# Autodesk Inventor assembly: aftServoSectionAssembly0
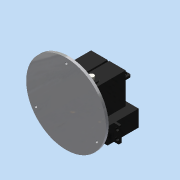
[picture p0: Inventor's stored thumbnail of the model, 180x180]
Saved by Autodesk Inventor 2017 (Build 210142000, 142)
## iProperties
Created: 2016-10-29
Part Number: aftServoSectionAssembly0
Document SubType Name: Assembly
Designer: techn
Author: techn
## Documents named in this file (4)
- D:\OneDrive\Documents\Other Projects\Submarine\CAD\midships\AftServoSection\aftServoSectionAssembly0.iam
- D:\OneDrive\Documents\Other Projects\Submarine\CAD\midships\AftServoSection\rearServoAttachmentPlate.ipt
- D:\OneDrive\Documents\Other Projects\Submarine\CAD\common\HitecServo\HitecServoAssembly.iam
- D:\OneDrive\Documents\Other Projects\Submarine\CAD\midships\AftServoSection\frontServoAttachmentPlate.ipt
## Components (5 placed, 3 different names)
1. rearServoAttachmentPlate:1 — Mate:1, Mate:2, Mate:3, Mate:4, Mate:5, Mate:6, Mate:7
2. HitecServoAssembly:1 [sub-assembly] — Mate:2, Mate:3, Mate:6, Mate:8, Flush:1, Mate:10, Mate:11
3. HitecServoAssembly:2 [sub-assembly] — Mate:1, Mate:4, Mate:5, Mate:9
4. HitecServoAssembly:3 [sub-assembly] — Mate:7, Mate:8, Flush:1
5. frontServoAttachmentPlate:1 — Mate:9, Mate:10, Mate:11
## Relationships (12: Mate 11, Flush 1)
- Mate:1: rearServoAttachmentPlate:1 ↔ HitecServoAssembly:2
- Mate:2: rearServoAttachmentPlate:1 ↔ HitecServoAssembly:1
- Mate:3: rearServoAttachmentPlate:1 ↔ HitecServoAssembly:1
- Mate:4: rearServoAttachmentPlate:1 ↔ HitecServoAssembly:2
- Mate:5: rearServoAttachmentPlate:1 ↔ HitecServoAssembly:2
- Mate:6: rearServoAttachmentPlate:1 ↔ HitecServoAssembly:1
- Mate:7: rearServoAttachmentPlate:1 ↔ HitecServoAssembly:3
- Mate:8 (1.27 mm): HitecServoAssembly:1 ↔ HitecServoAssembly:3
- Flush:1 (9.525 mm): HitecServoAssembly:1 ↔ HitecServoAssembly:3
- Mate:9: HitecServoAssembly:2 ↔ frontServoAttachmentPlate:1
- Mate:10: HitecServoAssembly:1 ↔ frontServoAttachmentPlate:1
- Mate:11: HitecServoAssembly:1 ↔ frontServoAttachmentPlate:1
